# Autodesk Inventor assembly: support orangepi
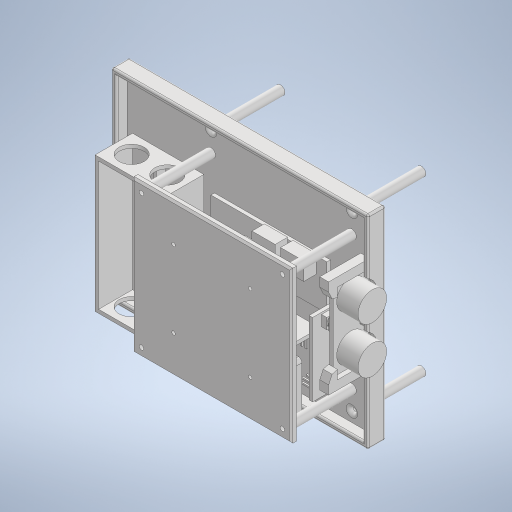
[picture p0: Inventor's stored thumbnail of the model, 512x512]
Saved by Autodesk Inventor 2024 (Build 280153000, 153)
## iProperties
Created: 2024-03-12
Part Number: support orangepi
Document SubType Name: Assembly
Designer: phaly
Author: phaly
## Documents named in this file (12)
- C:\Users\phaly\Music\Perso\Projet voiture\3D\Support\support orangepi.iam
- C:\Users\phaly\Music\Perso\Projet voiture\3D\Support\support.ipt
- C:\Users\phaly\Music\Perso\Projet voiture\3D\Support\support pile.ipt
- C:\Users\phaly\Music\Perso\Projet voiture\3D\Support\OrangePi.ipt
- C:\Users\phaly\Music\Perso\Projet voiture\3D\Support\Power.ipt
- C:\Users\phaly\Music\Perso\Projet voiture\3D\Support\convertisseur.ipt
- C:\Users\phaly\Music\Perso\Projet voiture\3D\Support\nrf24.ipt
- C:\Users\phaly\Music\Perso\Projet voiture\3D\Support\distance.ipt
- C:\Users\phaly\Music\Perso\Projet voiture\3D\Support\gyro.ipt
- C:\Users\phaly\Music\Perso\Projet voiture\3D\Support\cale.ipt
- C:\Users\phaly\Music\Perso\Projet voiture\3D\Support\support lidar.ipt
- C:\Users\phaly\Music\Perso\Projet voiture\3D\Support\elevateur support.ipt
## Components (19 placed, 11 different names)
1. support:1 — Placage:2, Placage:3, Placage:4, Placage:5, Placage:8, Placage:11, Placage:17, Placage:18, Placage:19, Placage:20, Placage:25, Placage:28, Placage:29, Placage:30, Placage:31, Placage:32, Placage:33, Placage:36, Placage:39, Placage:40, Placage:41, Placage:42, Placage:43, Placage:57, Placage:58, Placage:59, Placage:61, Placage:62, Placage:63, Placage:65
2. support pile:1 — Placage:2, Placage:3, Placage:4
3. OrangePi:1 — Placage:5, Placage:18, Placage:19, Affleurement:3, Placage:66, Affleurement:4
4. Power:1 — Placage:8, Placage:17, Placage:20
5. convertisseur:1 — Placage:11, Placage:25, Affleurement:3
6. distance:1 — Placage:32, Placage:33, Placage:34, Placage:35, Placage:37, Placage:38
7. nrf24:1 — Placage:29, Placage:30, Placage:31
8. gyro:1 — Placage:28, Placage:66, Affleurement:4
9. cale:1 — Placage:34, Placage:35, Placage:36
10. cale:2 — Placage:37, Placage:38, Placage:39
11. support lidar:1 — Placage:48, Placage:49, Placage:50, Placage:51, Placage:52, Placage:53, Placage:55, Placage:64
12. elevateur support:1 — Placage:40, Placage:62
13. elevateur support:2 — Placage:41, Placage:65
14. elevateur support:3 — Placage:42, Placage:61
15. elevateur support:4 — Placage:43, Placage:63
16. elevateur support:5 — Placage:49, Placage:59, Placage:64
17. elevateur support:6 — Placage:50, Placage:53, Placage:57
18. elevateur support:7 — Placage:48, Placage:55, Placage:58
19. elevateur support:8 — Placage:51, Placage:52
## Relationships (45: Mate 43, Flush 2)
- Placage:2 [Mate]: support:1 ↔ support pile:1
- Placage:3 [Mate] (3 mm): support:1 ↔ support pile:1
- Placage:4 [Mate] (3 mm): support:1 ↔ support pile:1
- Placage:5 [Mate] (18 mm): support:1 ↔ OrangePi:1
- Placage:8 [Mate]: support:1 ↔ Power:1
- Placage:11 [Mate]: support:1 ↔ convertisseur:1
- Placage:17 [Mate] (35 mm): support:1 ↔ Power:1
- Placage:18 [Mate] (5 mm): support:1 ↔ OrangePi:1
- Placage:19 [Mate] (22 mm): support:1 ↔ OrangePi:1
- Placage:20 [Mate] (24 mm): support:1 ↔ Power:1
- Placage:25 [Mate]: support:1 ↔ convertisseur:1
- Affleurement:3 [Flush]: OrangePi:1 ↔ convertisseur:1
- Placage:28 [Mate]: support:1 ↔ gyro:1
- Placage:29 [Mate]: support:1 ↔ nrf24:1
- Placage:30 [Mate] (15 mm): support:1 ↔ nrf24:1
- Placage:31 [Mate] (18 mm): support:1 ↔ nrf24:1
- Placage:32 [Mate]: support:1 ↔ distance:1
- Placage:33 [Mate]: support:1 ↔ distance:1
- Placage:34 [Mate]: distance:1 ↔ cale:1
- Placage:35 [Mate]: distance:1 ↔ cale:1
- Placage:36 [Mate]: support:1 ↔ cale:1
- Placage:37 [Mate]: distance:1 ↔ cale:2
- Placage:38 [Mate]: distance:1 ↔ cale:2
- Placage:39 [Mate]: support:1 ↔ cale:2
- Placage:40 [Mate]: support:1 ↔ elevateur support:1
- Placage:41 [Mate]: support:1 ↔ elevateur support:2
- Placage:42 [Mate]: support:1 ↔ elevateur support:3
- Placage:43 [Mate]: support:1 ↔ elevateur support:4
- Placage:48 [Mate]: support lidar:1 ↔ elevateur support:7
- Placage:49 [Mate]: support lidar:1 ↔ elevateur support:5
- Placage:50 [Mate]: support lidar:1 ↔ elevateur support:6
- Placage:51 [Mate]: support lidar:1 ↔ elevateur support:8
- Placage:52 [Mate]: support lidar:1 ↔ elevateur support:8
- Placage:53 [Mate]: support lidar:1 ↔ elevateur support:6
- Placage:55 [Mate]: support lidar:1 ↔ elevateur support:7
- Placage:57 [Mate]: support:1 ↔ elevateur support:6
- Placage:58 [Mate]: support:1 ↔ elevateur support:7
- Placage:59 [Mate]: support:1 ↔ elevateur support:5
- Placage:61 [Mate]: support:1 ↔ elevateur support:3
- Placage:62 [Mate]: support:1 ↔ elevateur support:1
- Placage:63 [Mate]: support:1 ↔ elevateur support:4
- Placage:64 [Mate]: support lidar:1 ↔ elevateur support:5
- Placage:65 [Mate]: support:1 ↔ elevateur support:2
- Placage:66 [Mate]: OrangePi:1 ↔ gyro:1
- Affleurement:4 [Flush]: OrangePi:1 ↔ gyro:1
